# Autodesk Inventor assembly: Assembly2
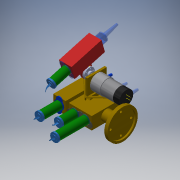
[picture p0: Inventor's stored thumbnail of the model, 180x180]
Saved by Autodesk Inventor 2018 (Build 220112000, 112)
## iProperties
Created: 2020-04-07
Part Number: Assembly2
Document SubType Name: Assembly
Designer: Jesse R-B
Author: Jesse R-B
## Documents named in this file (8)
- C:\Users\Jesse R-B\Documents\Inventor\400\V2\V3\Assembly2.iam
- C:\Users\Jesse R-B\Documents\Inventor\400\V2\V3\fingers1.ipt
- C:\Users\Jesse R-B\Documents\Inventor\400\Gearmotor_37D_100.ipt
- C:\Users\Jesse R-B\Documents\Inventor\400\pololu-universal-aluminum-mounting-hub-for-6mm-shaft-4-40-holes.ipt
- C:\Users\Jesse R-B\Documents\Inventor\400\V2\V3\thumb mount.ipt
- C:\Users\Jesse R-B\Documents\Inventor\400\V2\thumb.ipt
- C:\Users\Jesse R-B\Documents\Inventor\400\V2\syringeAssem.iam
- C:\Users\Jesse R-B\Documents\Inventor\400\V2\clawV2.ipt
## Components (13 placed, 7 different names)
1. fingers1:1 — Mate:1, Mate:2, Mate:3, Mate:9, Mate:10, Mate:11, Mate:14, Mate:15, Mate:16
2. Gearmotor_37D_100:1 — Mate:1, Mate:2, Mate:3, Mate:4, Flush:1
3. pololu-universal-aluminum-mounting-hub-for-6mm-shaft-4-40-holes:1 — Mate:4, Flush:1, Mate:5, Mate:6, Mate:7
4. thumb mount:1 — Mate:5, Mate:6, Mate:7, Flush:2, Flush:3, Mate:8
5. thumb:1 — Flush:2, Flush:3, Mate:8, Mate:12, Mate:13
6. syringeAssem:1 [sub-assembly] — Mate:9, Mate:16, Mate:19, Mate:22
7. syringeAssem:2 [sub-assembly] — Mate:10, Mate:15, Mate:20, Mate:21
8. syringeAssem:3 [sub-assembly] — Mate:11, Mate:14, Mate:17, Mate:18
9. syringeAssem:4 [sub-assembly] — Mate:12, Mate:13, Mate:23, Mate:24
10. clawV2:1 — Mate:23, Mate:24
11. clawV2:2 — Mate:19, Mate:22
12. clawV2:3 — Mate:17, Mate:18
13. clawV2:4 — Mate:20, Mate:21
## Relationships (27: Mate 24, Flush 3)
- Mate:1: fingers1:1 ↔ Gearmotor_37D_100:1
- Mate:2: fingers1:1 ↔ Gearmotor_37D_100:1
- Mate:3: fingers1:1 ↔ Gearmotor_37D_100:1
- Mate:4: Gearmotor_37D_100:1 ↔ pololu-universal-aluminum-mounting-hub-for-6mm-shaft-4-40-holes:1
- Flush:1: Gearmotor_37D_100:1 ↔ pololu-universal-aluminum-mounting-hub-for-6mm-shaft-4-40-holes:1
- Mate:5: pololu-universal-aluminum-mounting-hub-for-6mm-shaft-4-40-holes:1 ↔ thumb mount:1
- Mate:6: pololu-universal-aluminum-mounting-hub-for-6mm-shaft-4-40-holes:1 ↔ thumb mount:1
- Mate:7: pololu-universal-aluminum-mounting-hub-for-6mm-shaft-4-40-holes:1 ↔ thumb mount:1
- Flush:2: thumb mount:1 ↔ thumb:1
- Flush:3: thumb mount:1 ↔ thumb:1
- Mate:8: thumb mount:1 ↔ thumb:1
- Mate:9: fingers1:1 ↔ syringeAssem:1
- Mate:10: fingers1:1 ↔ syringeAssem:2
- Mate:11: fingers1:1 ↔ syringeAssem:3
- Mate:12: thumb:1 ↔ syringeAssem:4
- Mate:13: thumb:1 ↔ syringeAssem:4
- Mate:14: fingers1:1 ↔ syringeAssem:3
- Mate:15: fingers1:1 ↔ syringeAssem:2
- Mate:16: fingers1:1 ↔ syringeAssem:1
- Mate:17: syringeAssem:3 ↔ clawV2:3
- Mate:18: syringeAssem:3 ↔ clawV2:3
- Mate:19: syringeAssem:1 ↔ clawV2:2
- Mate:20: syringeAssem:2 ↔ clawV2:4
- Mate:21: syringeAssem:2 ↔ clawV2:4
- Mate:22: syringeAssem:1 ↔ clawV2:2
- Mate:23: syringeAssem:4 ↔ clawV2:1
- Mate:24: syringeAssem:4 ↔ clawV2:1
